# Autodesk Inventor assembly: Toaster
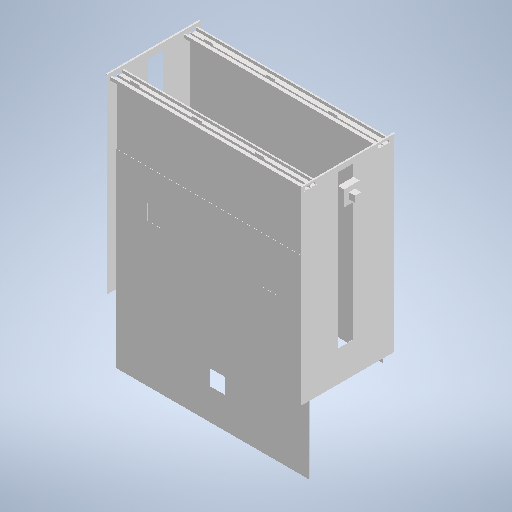
[picture p0: Inventor's stored thumbnail of the model, 512x512]
Saved by Autodesk Inventor 2025.1 (Build 291241020, 241B)
## iProperties
Created: 2024-09-24
Part Number: Toaster
Document SubType Name: Assembly
Designer: jjk
Author: jjk
## Documents named in this file (6)
- C:\Users\jjk\Desktop\Capstone CAD\Toaster.iam
- C:\Users\jjk\Desktop\Capstone CAD\Front Back side.ipt
- C:\Users\jjk\Desktop\Capstone CAD\Bracket holder.ipt
- C:\Users\jjk\Desktop\Capstone CAD\Heat sheild.ipt
- C:\Users\jjk\Desktop\Capstone CAD\Sensor board.ipt
- C:\Users\jjk\Desktop\Capstone CAD\Handle.ipt
## Components (8 placed, 5 different names)
1. Front Back side:1 — Mate:4, Mate:5, Mate:6, Mate:10
2. Front Back side:2 — Mate:1, Mate:2, Mate:3, Mate:7, Mate:8, Mate:13, Mate:15, Mate:16, Mate:18
3. Bracket holder:1 — Mate:1, Mate:2, Mate:3, Mate:4, Mate:5, Mate:6, Mate:11, Mate:12
4. Bracket holder:2 — Mate:7, Mate:8, Mate:10, Mate:17
5. Heat sheild:1 — Mate:11, Mate:12, Mate:14
6. Sensor board:1 — Mate:13, Mate:14
7. Handle:1 — Mate:15, Mate:16
8. Heat sheild:2 — Mate:17, Mate:18
## Relationships (17: Mate 17)
- Mate:1: Front Back side:2 ↔ Bracket holder:1
- Mate:2: Front Back side:2 ↔ Bracket holder:1
- Mate:3: Front Back side:2 ↔ Bracket holder:1
- Mate:4: Front Back side:1 ↔ Bracket holder:1
- Mate:5: Front Back side:1 ↔ Bracket holder:1
- Mate:6: Front Back side:1 ↔ Bracket holder:1
- Mate:7: Front Back side:2 ↔ Bracket holder:2
- Mate:8: Front Back side:2 ↔ Bracket holder:2
- Mate:10: Front Back side:1 ↔ Bracket holder:2
- Mate:11: Bracket holder:1 ↔ Heat sheild:1
- Mate:12: Bracket holder:1 ↔ Heat sheild:1
- Mate:13: Front Back side:2 ↔ Sensor board:1
- Mate:14: Heat sheild:1 ↔ Sensor board:1
- Mate:15: Front Back side:2 ↔ Handle:1
- Mate:16: Front Back side:2 ↔ Handle:1
- Mate:17: Bracket holder:2 ↔ Heat sheild:2
- Mate:18: Front Back side:2 ↔ Heat sheild:2
